# Autodesk Inventor assembly: F_Foot_v2
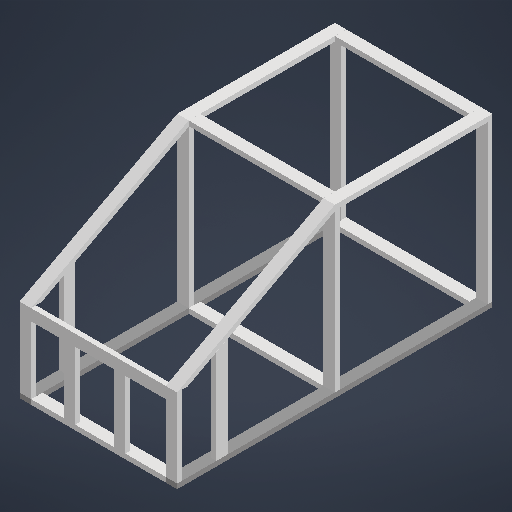
[picture p0: Inventor's stored thumbnail of the model, 512x512]
Saved by Autodesk Inventor 2027.1 (Build 311270010, 270A)
## iProperties
Created: 2026-08-30
Part Number: F_Foot_v2
Document SubType Name: Assembly
Designer: jorda
Author: jorda
## Documents named in this file (9)
- C:\Users\jorda\OneDrive\Documents\GitHub\USC-ASME-TigerBurn-2026\CAD\Legs\Front Foot\F_Foot_v2.iam
- C:\Users\jorda\OneDrive\Documents\GitHub\USC-ASME-TigerBurn-2026\CAD\Legs\Front Foot\2x4x48.ipt
- C:\Users\jorda\OneDrive\Documents\GitHub\USC-ASME-TigerBurn-2026\CAD\Legs\Front Foot\2x4x120.ipt
- C:\Users\jorda\OneDrive\Documents\GitHub\USC-ASME-TigerBurn-2026\CAD\Legs\Front Foot\2x4x41.ipt
- C:\Users\jorda\OneDrive\Documents\GitHub\USC-ASME-TigerBurn-2026\CAD\Legs\Front Foot\2x4x30.ipt
- C:\Users\jorda\OneDrive\Documents\GitHub\USC-ASME-TigerBurn-2026\CAD\Legs\Front Foot\2x4x96.ipt
- C:\Users\jorda\OneDrive\Documents\GitHub\USC-ASME-TigerBurn-2026\CAD\Legs\Front Foot\S_2x4x54.35.ipt
- C:\Users\jorda\OneDrive\Documents\GitHub\USC-ASME-TigerBurn-2026\CAD\Legs\Front Foot\S_2x4x30.5.ipt
- C:\Users\jorda\OneDrive\Documents\GitHub\USC-ASME-TigerBurn-2026\CAD\Legs\Front Foot\2x4x20.5.ipt
## Components (24 placed, 8 different names)
1. 2x4x120:1 — Mate:5, Flush:9, Flush:10, Mate:6, Flush:11, Flush:12, Flush:31, Mate:16, Flush:32, Flush:38, Flush:39
2. 2x4x48:2 — Mate:5, Flush:9, Flush:10, Mate:10, Flush:19, Flush:20
3. 2x4x120:2 — Mate:7, Flush:13, Flush:14, Mate:8, Flush:15, Flush:16, Mate:15, Flush:29, Mate:17, Flush:33, Flush:34
4. 2x4x48:3 — Mate:8, Flush:15, Flush:16, Mate:9, Flush:17, Flush:18, Mate:27, Flush:48, Flush:49
5. 2x4x41:1 — Mate:6, Flush:11, Flush:12, Flush:55, Flush:56, Mate:34
6. 2x4x41:2 — Mate:7, Flush:13, Flush:14, Flush:38, Flush:39
7. 2x4x48:4 — Mate:9, Flush:17, Flush:18, Mate:11, Flush:21, Flush:22, Mate:12, Flush:23, Flush:24, Mate:13, Flush:25, Flush:26, Mate:29
8. 2x4x48:5 — Mate:10, Flush:19, Flush:20, Mate:14, Flush:27, Flush:28, Mate:30, Flush:53
9. 2x4x41:3 — Mate:11, Flush:21, Flush:22
10. 2x4x41:4 — Mate:12, Flush:23, Flush:24
11. 2x4x48:6 — Mate:13, Flush:25, Flush:26, Flush:30, Flush:52
12. 2x4x48:7 — Mate:14, Flush:27, Flush:28
13. 2x4x41:5 — Mate:15, Flush:29, Flush:30
14. 2x4x30:1 — Flush:31, Mate:16, Flush:32, Mate:23, Mate:28, Flush:50, Flush:51
15. 2x4x30:2 — Mate:17, Flush:33, Flush:34, Flush:43, Flush:57, Mate:35
16. 2x4x41:7 — Flush:43, Mate:23, Mate:64, Flush:74, Mate:65, Flush:75
17. 2x4x96:1 — Mate:27, Flush:48, Flush:49, Flush:57, Mate:35, Mate:60, Flush:69
18. 2x4x96:2 — Mate:28, Flush:50, Flush:51, Flush:55, Flush:56, Mate:34, Mate:61, Flush:71
19. S_2x4x54.35:1 — Mate:29, Flush:52
20. S_2x4x54.35:2 — Mate:30, Flush:53
21. S_2x4x30.5:1 — Mate:60, Flush:69, Flush:70
22. S_2x4x30.5:2 — Mate:61, Flush:70, Flush:71
23. 2x4x20.5:2 — Mate:64, Flush:74
24. 2x4x20.5:3 — Mate:65, Flush:75
## Relationships (67: Flush 43, Mate 24)
- Mate:5: 2x4x120:1 ↔ 2x4x48:2
- Flush:9: 2x4x120:1 ↔ 2x4x48:2
- Flush:10: 2x4x120:1 ↔ 2x4x48:2
- Mate:6: 2x4x120:1 ↔ 2x4x41:1
- Flush:11: 2x4x120:1 ↔ 2x4x41:1
- Flush:12: 2x4x120:1 ↔ 2x4x41:1
- Mate:7: 2x4x120:2 ↔ 2x4x41:2
- Flush:13: 2x4x120:2 ↔ 2x4x41:2
- Flush:14: 2x4x120:2 ↔ 2x4x41:2
- Mate:8: 2x4x120:2 ↔ 2x4x48:3
- Flush:15: 2x4x120:2 ↔ 2x4x48:3
- Flush:16: 2x4x120:2 ↔ 2x4x48:3
- Mate:9: 2x4x48:3 ↔ 2x4x48:4
- Flush:17: 2x4x48:3 ↔ 2x4x48:4
- Flush:18: 2x4x48:3 ↔ 2x4x48:4
- Mate:10: 2x4x48:2 ↔ 2x4x48:5
- Flush:19: 2x4x48:2 ↔ 2x4x48:5
- Flush:20: 2x4x48:2 ↔ 2x4x48:5
- Mate:11: 2x4x48:4 ↔ 2x4x41:3
- Flush:21: 2x4x48:4 ↔ 2x4x41:3
- Flush:22: 2x4x48:4 ↔ 2x4x41:3
- Mate:12: 2x4x48:4 ↔ 2x4x41:4
- Flush:23: 2x4x48:4 ↔ 2x4x41:4
- Flush:24: 2x4x48:4 ↔ 2x4x41:4
- Mate:13: 2x4x48:4 ↔ 2x4x48:6
- Flush:25: 2x4x48:4 ↔ 2x4x48:6
- Flush:26: 2x4x48:4 ↔ 2x4x48:6
- Mate:14: 2x4x48:5 ↔ 2x4x48:7
- Flush:27: 2x4x48:5 ↔ 2x4x48:7
- Flush:28: 2x4x48:5 ↔ 2x4x48:7
- Mate:15: 2x4x120:2 ↔ 2x4x41:5
- Flush:29: 2x4x120:2 ↔ 2x4x41:5
- Flush:30: 2x4x48:6 ↔ 2x4x41:5
- Flush:31: 2x4x120:1 ↔ 2x4x30:1
- Mate:16: 2x4x120:1 ↔ 2x4x30:1
- Flush:32: 2x4x120:1 ↔ 2x4x30:1
- Mate:17: 2x4x120:2 ↔ 2x4x30:2
- Flush:33: 2x4x120:2 ↔ 2x4x30:2
- Flush:34: 2x4x120:2 ↔ 2x4x30:2
- Flush:38: 2x4x120:1 ↔ 2x4x41:2
- Flush:39: 2x4x120:1 ↔ 2x4x41:2
- Flush:43: 2x4x30:2 ↔ 2x4x41:7
- Mate:23: 2x4x30:1 ↔ 2x4x41:7
- Mate:27: 2x4x48:3 ↔ 2x4x96:1
- Flush:48: 2x4x48:3 ↔ 2x4x96:1
- Flush:49: 2x4x48:3 ↔ 2x4x96:1
- Mate:28: 2x4x30:1 ↔ 2x4x96:2
- Flush:50: 2x4x30:1 ↔ 2x4x96:2
- Flush:51: 2x4x30:1 ↔ 2x4x96:2
- Mate:29: 2x4x48:4 ↔ S_2x4x54.35:1
- Flush:52: 2x4x48:6 ↔ S_2x4x54.35:1
- Mate:30: 2x4x48:5 ↔ S_2x4x54.35:2
- Flush:53: 2x4x48:5 ↔ S_2x4x54.35:2
- Flush:55: 2x4x41:1 ↔ 2x4x96:2
- Flush:56: 2x4x41:1 ↔ 2x4x96:2
- Mate:34: 2x4x41:1 ↔ 2x4x96:2
- Flush:57: 2x4x30:2 ↔ 2x4x96:1
- Mate:35: 2x4x30:2 ↔ 2x4x96:1
- Mate:60: 2x4x96:1 ↔ S_2x4x30.5:1
- Flush:69: 2x4x96:1 ↔ S_2x4x30.5:1
- Mate:61: 2x4x96:2 ↔ S_2x4x30.5:2
- Flush:70: S_2x4x30.5:1 ↔ S_2x4x30.5:2
- Flush:71: 2x4x96:2 ↔ S_2x4x30.5:2
- Mate:64: 2x4x41:7 ↔ 2x4x20.5:2
- Flush:74: 2x4x41:7 ↔ 2x4x20.5:2
- Mate:65: 2x4x41:7 ↔ 2x4x20.5:3
- Flush:75: 2x4x41:7 ↔ 2x4x20.5:3
